# Autodesk Inventor assembly: polia+rolamento-no-centro
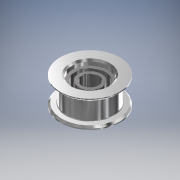
[picture p0: Inventor's stored thumbnail of the model, 180x180]
Saved by Autodesk Inventor 2017 SP1 (Build 210196100, 196)
## iProperties
Created: 2016-07-27
Part Number: polia+rolamento-no-centro
Document SubType Name: Assembly
Designer: Henrique Miguel
Author: Henrique Miguel
## Documents named in this file (3)
- K:\Dropbox\Mecânica\Suprimentos\Polias\polia+rolamento-no-centro.iam
- K:\Dropbox\Mecânica\Suprimentos\Usinados\PoliaLisaGT2.ipt
- K:\Dropbox\Mecânica\Suprimentos\Rolamentos\ROL.RAD.D05XD11X5.ipt
## Components (2 placed, 2 different names)
1. PoliaLisaGT2:1 — Rigid:1
2. Bearing GB/T 5800-2003 638/5:2 — Rigid:1
## Relationships (1: WeldJoint 1)
- Rigid:1 [WeldJoint]: PoliaLisaGT2:1 ↔ Bearing GB/T 5800-2003 638/5:2
